# Autodesk Inventor assembly: BV-ASM-222-105
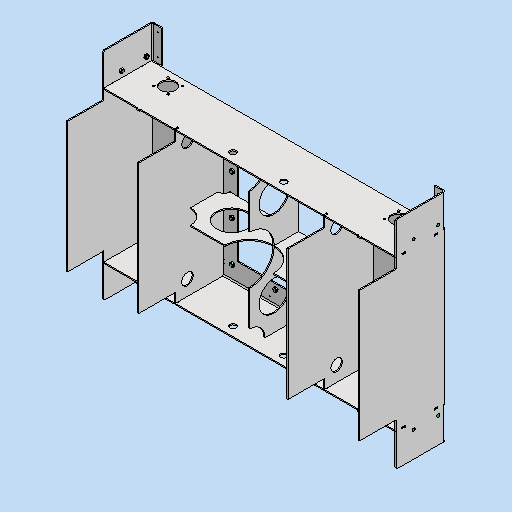
[picture p0: Inventor's stored thumbnail of the model, 512x512]
Saved by Autodesk Inventor 2025.3 (Build 293356030, 356C)
## iProperties
Created: 2025-12-10
Part Number: BV-ASM-222-105
Document SubType Name: Assembly
Designer: josh
Mass: 79753.3 g
Surface Area: 44003 cm^2
Volume: 10159.7 cm^3
Density: 7.85 g/cm^3
Description: BASE WELDMENT STEP ONE
Author: josh
## Documents named in this file (7)
- R:\A1- Neuweg Design Data\OM Robotics\BASE VEHICLE DESIGN PROJECT\BV-ASM-222-105.iam
- R:\A1- Neuweg Design Data\OM Robotics\BASE VEHICLE DESIGN PROJECT\BV-222-102.ipt
- R:\A1- Neuweg Design Data\OM Robotics\BASE VEHICLE DESIGN PROJECT\BV-222-104.ipt
- R:\A1- Neuweg Design Data\OM Robotics\BASE VEHICLE DESIGN PROJECT\BV-222-110.ipt
- R:\A1- Neuweg Design Data\OM Robotics\BASE VEHICLE DESIGN PROJECT\BV-222-111.ipt
- R:\A1- Neuweg Design Data\OM Robotics\BASE VEHICLE DESIGN PROJECT\93560A112.ipt
- R:\A1- Neuweg Design Data\OM Robotics\BASE VEHICLE DESIGN PROJECT\BV-222-103.ipt
## Components (27 placed, 6 different names)
1. BV-222-102:1 — Mate:1, Mate:2, Flush:1, Flush:2, Flush:3, Flush:4
2. BV-222-104:2
3. BV-222-104:1
4. BV-222-111:1
5. BV-222-110:1
6. 93560A112:1
7. 93560A112:2
8. 93560A112:3
9. 93560A112:4
10. 93560A112:5
11. 93560A112:6
12. 93560A112:7
13. 93560A112:8
14. 93560A112:9
15. 93560A112:10
16. 93560A112:11
17. 93560A112:12
18. BV-222-103:2 — Insert:3, Flush:2, Flush:3, Flush:4, Insert:6, Insert:7, Insert:8
19. BV-222-103:1 — Insert:1, Insert:2, Insert:4, Mate:1, Mate:2, Flush:1, Insert:5
20. 93560A112:17 — Insert:2
21. 93560A112:18 — Insert:1
22. 93560A112:19 — Insert:3
23. 93560A112:20 — Insert:4
24. 93560A112:21 — Insert:5
25. 93560A112:22 — Insert:7
26. 93560A112:23 — Insert:6
27. 93560A112:24 — Insert:8
## Relationships (14: Insert 8, Flush 4, Mate 2)
- Insert:1: BV-222-103:1 ↔ 93560A112:18
- Insert:2: BV-222-103:1 ↔ 93560A112:17
- Insert:3: BV-222-103:2 ↔ 93560A112:19
- Insert:4: BV-222-103:1 ↔ 93560A112:20
- Mate:1: BV-222-102:1 ↔ BV-222-103:1
- Mate:2: BV-222-102:1 ↔ BV-222-103:1
- Flush:1: BV-222-102:1 ↔ BV-222-103:1
- Flush:2: BV-222-102:1 ↔ BV-222-103:2
- Flush:3: BV-222-102:1 ↔ BV-222-103:2
- Flush:4: BV-222-102:1 ↔ BV-222-103:2
- Insert:5: BV-222-103:1 ↔ 93560A112:21
- Insert:6: BV-222-103:2 ↔ 93560A112:23
- Insert:7: BV-222-103:2 ↔ 93560A112:22
- Insert:8: BV-222-103:2 ↔ 93560A112:24
## Named parameters: d29_d142 = 0 mm, d30_d118 = 0 mm, d31_d124 = 0 mm, d32_d140 = 0 mm
